# Autodesk Inventor assembly: Inner_Components
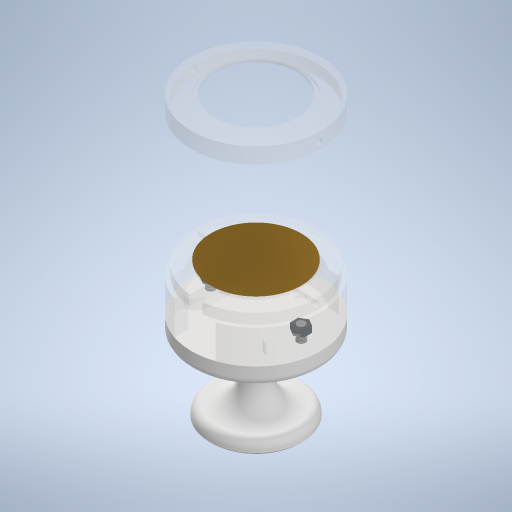
[picture p0: Inventor's stored thumbnail of the model, 512x512]
Saved by Autodesk Inventor 2023 (Build 270158000, 158)
## iProperties
Created: 2023-02-27
Part Number: Inner_Components
Document SubType Name: Assembly
Designer: maste
Author: maste
## Documents named in this file (7)
- C:\Users\maste\Documents\GitHub\Remote-Stethoscope\3D_models\ThonkLabs 1ne\SurfaceContact\Inner_Components.iam
- C:\Users\maste\Documents\GitHub\Remote-Stethoscope\3D_models\ThonkLabs 1ne\SurfaceContact\PiezoMount.ipt
- C:\Users\maste\Documents\GitHub\Remote-Stethoscope\3D_models\ThonkLabs 1ne\SurfaceContact\Piezo.ipt
- C:\Users\maste\Documents\GitHub\Remote-Stethoscope\3D_models\ThonkLabs 1ne\SurfaceContact\Diaphragm_lock.ipt
- C:\Users\maste\Documents\GitHub\Remote-Stethoscope\3D_models\ThonkLabs 1ne\SurfaceContact\holding_socket.ipt
- C:\Users\maste\Documents\GitHub\Remote-Stethoscope\3D_models\ThonkLabs 1ne\SurfaceContact\fasten_nut.ipt
- C:\Users\maste\Documents\GitHub\Remote-Stethoscope\3D_models\ThonkLabs 1ne\SurfaceContact\fasten_bolt.ipt
## Components (8 placed, 6 different names)
1. PiezoMount:1 — Mate:2, Mate:7, Mate:8, Mate:9, Mate:10, Mate:11, Mate:12, Mate:14, Mate:15, Mate:16, Mate:17
2. Piezo:1 — Mate:2, Mate:12, Mate:13
3. Diaphragm_lock:1 — Mate:11, Mate:13
4. holding_socket:1 — Mate:7, Mate:8, Mate:9, Mate:10, Mate:18, Mate:19
5. fasten_nut:1 — Mate:14, Mate:15
6. fasten_nut:2 — Mate:16, Mate:17
7. fasten_bolt:1 — Mate:18
8. fasten_bolt:2 — Mate:19
## Relationships (14: Mate 14)
- Mate:2: PiezoMount:1 ↔ Piezo:1
- Mate:7: PiezoMount:1 ↔ holding_socket:1
- Mate:8: PiezoMount:1 ↔ holding_socket:1
- Mate:9: PiezoMount:1 ↔ holding_socket:1
- Mate:10: PiezoMount:1 ↔ holding_socket:1
- Mate:11: PiezoMount:1 ↔ Diaphragm_lock:1
- Mate:12: PiezoMount:1 ↔ Piezo:1
- Mate:13: Piezo:1 ↔ Diaphragm_lock:1
- Mate:14: PiezoMount:1 ↔ fasten_nut:1
- Mate:15: PiezoMount:1 ↔ fasten_nut:1
- Mate:16: PiezoMount:1 ↔ fasten_nut:2
- Mate:17: PiezoMount:1 ↔ fasten_nut:2
- Mate:18: holding_socket:1 ↔ fasten_bolt:1
- Mate:19: holding_socket:1 ↔ fasten_bolt:2
